# Autodesk Inventor assembly: Expansion_Module_PCB_Assembly
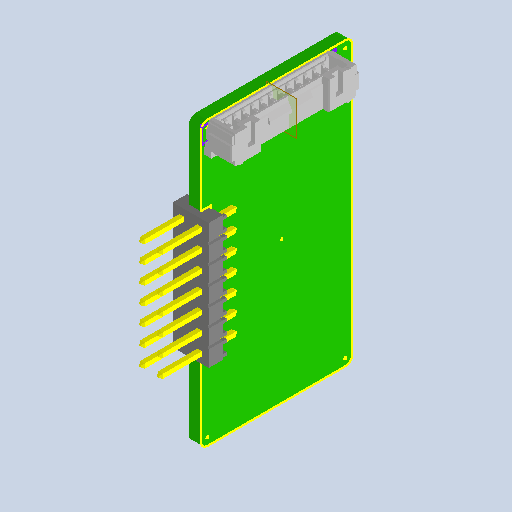
[picture p0: Inventor's stored thumbnail of the model, 512x512]
Saved by Autodesk Inventor 2024.2 (Build 282272000, 272)
## iProperties
Created: 2020-07-14
Part Number: Expansion_Module_PCB_Assembly
Document SubType Name: Assembly
Designer: CASE-SMALL2
Author: CASE-SMALL2
## Documents named in this file (4)
- C:\Users\lgnds\Documents\GitHub\REACH-Hardware\CAD\InventorProject\PCB_Assemblies\Expansion_Module_PCB_Assembly.iam
- C:\Users\lgnds\Documents\GitHub\REACH-Hardware\CAD\InventorProject\PCB_Assemblies\PCB\Expasion_Module_PCB.ipt
- C:\Users\lgnds\Documents\GitHub\REACH-Hardware\CAD\InventorProject\PCB_Assemblies\Connector\MOLEX 5055671231.ipt
- C:\Users\lgnds\Documents\GitHub\REACH-Hardware\CAD\InventorProject\PCB_Assemblies\Connector\TSW-107-07-G-D\TSW-107-07-G-D.iam
## Components (3 placed, 3 different names)
1. Expasion_Module_PCB:1 — Flush:1, Mate:1, Flush:2, Rigid:1
2. MOLEX 5055671231:1 — Flush:1, Mate:1, Flush:2
3. TSW-107-07-G-D:1 [sub-assembly] — Rigid:1
## Relationships (4: Flush 2, Mate 1, WeldJoint 1)
- Flush:1 (0.5 mm): Expasion_Module_PCB:1 ↔ MOLEX 5055671231:1
- Mate:1: Expasion_Module_PCB:1 ↔ MOLEX 5055671231:1
- Flush:2: Expasion_Module_PCB:1 ↔ MOLEX 5055671231:1
- Rigid:1 [WeldJoint]: Expasion_Module_PCB:1 ↔ TSW-107-07-G-D:1
